# Autodesk Inventor assembly: foot_MIR
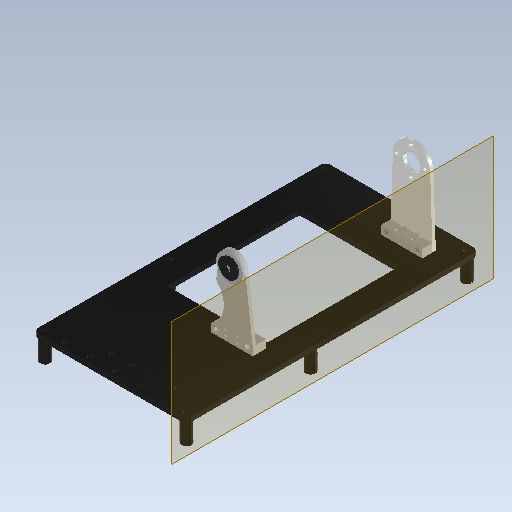
[picture p0: Inventor's stored thumbnail of the model, 512x512]
Saved by Autodesk Inventor 2020.4 (Build 244396000, 396)
## iProperties
Created: 2021-09-07
Part Number: foot_MIR
Document SubType Name: Assembly
Designer: Masato
Mass: 68.6803 g
Surface Area: 351.037 cm^2
Volume: 41.2832 cm^3
Density: 1.66364 g/cm^3
Title: Foot
Author: naoki
## Documents named in this file (9)
- C:\Users\Masato\Documents\Inventor\CIT Brains_Inventor\OpenPlatform_ver3_0\LowerBody\Foot\Foot_MIR.iam
- C:\Users\Masato\Documents\Inventor\CIT Brains_Inventor\OpenPlatform_ver3_0\LowerBody\Foot\sole.ipt
- C:\Users\Masato\Documents\Inventor\CIT Brains_Inventor\OpenPlatform_ver3_0\LowerBody\Foot\Foot_vertical_01.ipt
- C:\Users\Masato\Documents\Inventor\CIT Brains_Inventor\OpenPlatform_ver3_0\Ready_Made\ARU-313SMO.ipt
- C:\Users\Masato\Documents\Inventor\CIT Brains_Inventor\OpenPlatform_ver3_0\LowerBody\Foot\Foot_roll_vertical_02.ipt
- C:\Users\Masato\Documents\Inventor\CIT Brains_Inventor\OpenPlatform_ver3_0\LowerBody\Foot\Foot_roll_vertical_01.ipt
- C:\Users\Masato\Documents\Inventor\CIT Brains_Inventor\OpenPlatform_ver3_0\Ready_Made\80F-0603.ipt
- C:\Users\Masato\Documents\Inventor\CIT Brains_Inventor\OpenPlatform_ver3_0\Ready_Made\LFW-0815.ipt
- C:\Users\Masato\Documents\Inventor\CIT Brains_Inventor\OpenPlatform_ver3_0\Ready_Made\UUW-0312-10BH.ipt
## Components (14 placed, 8 different names)
1. sole:1 — メイト:3, メイト:2, メイト:1, 挿入:10, 挿入:9, 挿入:8, 挿入:7, 挿入:6, 挿入:5, 挿入:30, 挿入:31, 挿入:34, 挿入:35
2. Foot_vertical_01:1 — 挿入:30, 挿入:31, 挿入:38, 挿入:39
3. Foot_vertical_01:2 — 挿入:34, 挿入:35, 挿入:36, 挿入:37
4. ARU-313SMO:1 — 挿入:10
5. ARU-313SMO:2 — 挿入:9
6. ARU-313SMO:3 — 挿入:8
7. ARU-313SMO:4 — 挿入:7
8. ARU-313SMO:5 — 挿入:6
9. ARU-313SMO:6 — 挿入:5
10. Foot_roll_vertical_02:1 — 挿入:36, 挿入:37
11. Foot_roll_vertical_01:1 — 挿入:28, 挿入:29, 挿入:38, 挿入:39
12. 80F-0603:1 — 挿入:28
13. LFW-0815:1 — 挿入:18, 挿入:29
14. UUW-0312-10BH:1 — 挿入:18
## Relationships (20: Insert 17, Mate 3)
- メイト:3 [Mate]: sole:1
- メイト:2 [Mate]: sole:1
- メイト:1 [Mate]: sole:1
- 挿入:10 [Insert]: sole:1 ↔ ARU-313SMO:1
- 挿入:9 [Insert]: sole:1 ↔ ARU-313SMO:2
- 挿入:8 [Insert]: sole:1 ↔ ARU-313SMO:3
- 挿入:7 [Insert]: sole:1 ↔ ARU-313SMO:4
- 挿入:6 [Insert]: sole:1 ↔ ARU-313SMO:5
- 挿入:5 [Insert]: sole:1 ↔ ARU-313SMO:6
- 挿入:18 [Insert]: LFW-0815:1 ↔ UUW-0312-10BH:1
- 挿入:28 [Insert]: Foot_roll_vertical_01:1 ↔ 80F-0603:1
- 挿入:29 [Insert]: Foot_roll_vertical_01:1 ↔ LFW-0815:1
- 挿入:30 [Insert]: sole:1 ↔ Foot_vertical_01:1
- 挿入:31 [Insert]: sole:1 ↔ Foot_vertical_01:1
- 挿入:34 [Insert]: sole:1 ↔ Foot_vertical_01:2
- 挿入:35 [Insert]: sole:1 ↔ Foot_vertical_01:2
- 挿入:36 [Insert]: Foot_vertical_01:2 ↔ Foot_roll_vertical_02:1
- 挿入:37 [Insert]: Foot_vertical_01:2 ↔ Foot_roll_vertical_02:1
- 挿入:38 [Insert]: Foot_vertical_01:1 ↔ Foot_roll_vertical_01:1
- 挿入:39 [Insert]: Foot_vertical_01:1 ↔ Foot_roll_vertical_01:1
